# Autodesk Inventor assembly: Gripper_Mount
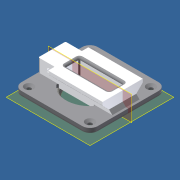
[picture p0: Inventor's stored thumbnail of the model, 180x180]
Saved by Autodesk Inventor 2014 SP2 (Build 180246200, 246)
## iProperties
Created: 2015-02-28
Part Number: Gripper_Mount
Document SubType Name: Assembly
Designer: 4ndreas
Author: 4ndreas
## Documents named in this file (3)
- C:\Users\4ndreas\Documents\Inventor\RobotARM v2\v3\Gripper_Mount.iam
- C:\Users\4ndreas\Documents\Inventor\RobotARM v2\70mmkugellager.ipt
- C:\Users\4ndreas\Documents\Inventor\RobotARM v2\v3\Gripper_Coupling.ipt
## Components (2 placed, 2 different names)
1. 70mmkugellager:1 — Passend:1, Passend:2, Winkel:1
2. Gripper_Coupling:1
## Relationships (3: Mate 2, Angle 1)
- Passend:1 [Mate]: 70mmkugellager:1
- Passend:2 [Mate]: 70mmkugellager:1
- Winkel:1 [Angle] (0 deg): 70mmkugellager:1
